# Autodesk Inventor assembly: frame
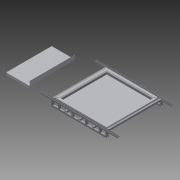
[picture p0: Inventor's stored thumbnail of the model, 180x180]
Saved by Autodesk Inventor 2013 (Build 170138000, 138)
## iProperties
Created: 2012-10-19
Part Number: frame
Document SubType Name: Assembly
Designer: Istvan
Author: Istvan
## Documents named in this file (5)
- D:\GitHub\Crown-Fire\CAD\Frame\frame.iam
- D:\GitHub\Crown-Fire\CAD\Frame\Table\table.iam
- D:\GitHub\Crown-Fire\CAD\Frame\Supports\supports.iam
- D:\GitHub\Crown-Fire\CAD\Frame\WorkTable\workTable.ipt
- D:\GitHub\Crown-Fire\CAD\Frame\Gantry\y-axisTrucks\rack.ipt
## Components (5 placed, 4 different names)
1. table:1 [sub-assembly] — Mate:1, Mate:2, Mate:5, Mate:6
2. supports:1 [sub-assembly] — Mate:1, Mate:2, Mate:3, Mate:4, Mate:5, Mate:6, Mate:7, Mate:8, Flush:1, Flush:2
3. workTable:1 — Mate:3, Mate:4
4. rack:1 — Mate:7, Flush:2
5. rack:2 — Mate:8, Flush:1
## Relationships (10: Mate 8, Flush 2)
- Mate:1 (12.7 mm): table:1 ↔ supports:1
- Mate:2 (12.7 mm): table:1 ↔ supports:1
- Mate:3: supports:1 ↔ workTable:1
- Mate:4: supports:1 ↔ workTable:1
- Mate:5: table:1 ↔ supports:1
- Mate:6 (6.35 mm): table:1 ↔ supports:1
- Mate:7: supports:1 ↔ rack:1
- Mate:8: supports:1 ↔ rack:2
- Flush:1: supports:1 ↔ rack:2
- Flush:2: supports:1 ↔ rack:1
